# Autodesk Inventor assembly: Head
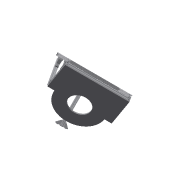
[picture p0: Inventor's stored thumbnail of the model, 180x180]
Saved by Autodesk Inventor 2014 SP1 (Build 180222100, 222)
## iProperties
Created: 2015-02-11
Part Number: Head
Document SubType Name: Assembly
Designer: Simen
Author: Simen
## Documents named in this file (9)
- C:\Users\Simen\Documents\git\Eit\skjellet\Head2.iam
- C:\Users\Simen\Documents\git\Eit\skjellet\HBL45TS6hbl45ts6.ipt
- C:\Users\Simen\Documents\git\Eit\skjellet\KHFS5_2020_386.ipt
- C:\Users\Simen\Documents\git\Eit\skjellet\KHFS5_2020_391.ipt
- C:\Users\Simen\Documents\git\Eit\skjellet\KHFS5_2020_220.ipt
- C:\Users\Simen\Documents\git\Eit\skjellet\frontPlate_half.ipt
- C:\Users\Simen\Documents\git\Eit\skjellet\jorneFester.iam
- C:\Users\Simen\Documents\git\Eit\skjellet\KHFS5_2020_426.ipt
- C:\Users\Simen\Documents\git\Eit\skjellet\KHFS5_2020_330.ipt
## Components (22 placed, 4 different names)
1. HBL45TS6hbl45ts6:2 — Mate:41, Flush:39, Mate:44, Mate:74, Mate:75, Flush:59
2. KHFS5-2020-4000:17 — Flush:64, Mate:83, Flush:65, Flush:66, Flush:67, Flush:68, Mate:84, Flush:83
3. KHFS5-2020-4000:18 — Mate:41, Flush:39, Mate:44, Mate:124, Flush:119, Flush:120, Mate:126, Flush:121
4. KHFS5-2020-4000:19 — Mate:81, Flush:63, Mate:82, Mate:116, Flush:115
5. KHFS5-2020-4000:34 — Mate:74, Mate:75, Flush:59, Flush:64, Flush:67, Flush:68, Mate:84, Flush:82, Mate:123, Mate:125
6. HBL45TS6hbl45ts6:3 — Mate:81, Flush:63
7. KHFS5-2020-4000:35 — Mate:82, Mate:83, Flush:65, Flush:66, Mate:93, Mate:117, Flush:116, Mate:119
8. frontPlate_half:1 — Mate:93, Flush:82, Flush:83
9. jorneFester:7 [sub-assembly] — Mate:129, Mate:131, Flush:124
10. jorneFester:5 [sub-assembly] — Mate:134, Mate:136, Flush:126, Flush:127, Flush:128, Mate:137, Flush:129
11. jorneFester:4 [sub-assembly] — Mate:128, Mate:132, Flush:123
12. jorneFester:2 [sub-assembly] — Mate:133, Mate:134, Flush:125, Flush:126, Mate:137, Mate:138
13. jorneFester:1 [sub-assembly] — Mate:133, Mate:135, Flush:127, Mate:139
14. jorneFester:3 [sub-assembly] — Mate:135, Mate:136, Flush:125, Flush:128
15. HBL45TS6hbl45ts6:4 — Mate:116, Flush:115
16. KHFS5-2020-4000:48 — Mate:118, Mate:119
17. jorneFester:8 [sub-assembly] — Mate:117, Flush:116, Mate:118
18. HBL45TS6hbl45ts6:5 — Mate:124, Flush:119
19. KHFS5-2020-4000:49 — Flush:118, Mate:125
20. jorneFester:9 [sub-assembly] — Mate:123, Flush:118
21. KHFS5-2020-4000:50 — Flush:120, Mate:126, Flush:121, Mate:128, Mate:129, Mate:130, Flush:122, Flush:123, Flush:124
22. KHFS5-2020-4000:51 — Mate:130, Flush:122, Mate:131, Mate:132, Mate:138, Mate:139, Flush:129
## Relationships (63: Mate 36, Flush 27)
- Mate:41: HBL45TS6hbl45ts6:2 ↔ KHFS5-2020-4000:18
- Flush:39: HBL45TS6hbl45ts6:2 ↔ KHFS5-2020-4000:18
- Mate:44: HBL45TS6hbl45ts6:2 ↔ KHFS5-2020-4000:18
- Mate:74: HBL45TS6hbl45ts6:2 ↔ KHFS5-2020-4000:34
- Mate:75: HBL45TS6hbl45ts6:2 ↔ KHFS5-2020-4000:34
- Flush:59: HBL45TS6hbl45ts6:2 ↔ KHFS5-2020-4000:34
- [Mate]: HBL45TS6hbl45ts6:3 ↔ KHFS5-2020-4000:35
- [Mate]: HBL45TS6hbl45ts6:3 ↔ KHFS5-2020-4000:35
- [Flush]: HBL45TS6hbl45ts6:3 ↔ KHFS5-2020-4000:35
- Mate:81: KHFS5-2020-4000:19 ↔ HBL45TS6hbl45ts6:3
- Flush:63: KHFS5-2020-4000:19 ↔ HBL45TS6hbl45ts6:3
- Mate:82: KHFS5-2020-4000:19 ↔ KHFS5-2020-4000:35
- Flush:64: KHFS5-2020-4000:17 ↔ KHFS5-2020-4000:34
- Mate:83: KHFS5-2020-4000:17 ↔ KHFS5-2020-4000:35
- Flush:65: KHFS5-2020-4000:17 ↔ KHFS5-2020-4000:35
- Flush:66: KHFS5-2020-4000:17 ↔ KHFS5-2020-4000:35
- Flush:67: KHFS5-2020-4000:17 ↔ KHFS5-2020-4000:34
- Flush:68: KHFS5-2020-4000:17 ↔ KHFS5-2020-4000:34
- Mate:84: KHFS5-2020-4000:17 ↔ KHFS5-2020-4000:34
- Mate:93: KHFS5-2020-4000:35 ↔ frontPlate_half:1
- Flush:82: KHFS5-2020-4000:34 ↔ frontPlate_half:1
- Flush:83: KHFS5-2020-4000:17 ↔ frontPlate_half:1
- [Mate]: HBL45TS6hbl45ts6:4 ↔ KHFS5-2020-4000:48
- [Mate]: HBL45TS6hbl45ts6:4 ↔ KHFS5-2020-4000:48
- [Flush]: HBL45TS6hbl45ts6:4 ↔ KHFS5-2020-4000:48
- Mate:116: KHFS5-2020-4000:19 ↔ HBL45TS6hbl45ts6:4
- Flush:115: KHFS5-2020-4000:19 ↔ HBL45TS6hbl45ts6:4
- Mate:117: KHFS5-2020-4000:35 ↔ jorneFester:8
- Flush:116: KHFS5-2020-4000:35 ↔ jorneFester:8
- Mate:118: KHFS5-2020-4000:48 ↔ jorneFester:8
- Mate:119: KHFS5-2020-4000:35 ↔ KHFS5-2020-4000:48
- [Mate]: HBL45TS6hbl45ts6:5 ↔ KHFS5-2020-4000:49
- [Mate]: HBL45TS6hbl45ts6:5 ↔ KHFS5-2020-4000:49
- [Flush]: HBL45TS6hbl45ts6:5 ↔ KHFS5-2020-4000:49
- [Mate]: KHFS5-2020-4000:49 ↔ jorneFester:9
- Mate:123: KHFS5-2020-4000:34 ↔ jorneFester:9
- Flush:118: KHFS5-2020-4000:49 ↔ jorneFester:9
- Mate:124: KHFS5-2020-4000:18 ↔ HBL45TS6hbl45ts6:5
- Flush:119: KHFS5-2020-4000:18 ↔ HBL45TS6hbl45ts6:5
- Mate:125: KHFS5-2020-4000:34 ↔ KHFS5-2020-4000:49
- Flush:120: KHFS5-2020-4000:18 ↔ KHFS5-2020-4000:50
- Mate:126: KHFS5-2020-4000:18 ↔ KHFS5-2020-4000:50
- Flush:121: KHFS5-2020-4000:18 ↔ KHFS5-2020-4000:50
- Mate:128: jorneFester:4 ↔ KHFS5-2020-4000:50
- Mate:129: jorneFester:7 ↔ KHFS5-2020-4000:50
- Mate:130: KHFS5-2020-4000:50 ↔ KHFS5-2020-4000:51
- Flush:122: KHFS5-2020-4000:50 ↔ KHFS5-2020-4000:51
- Mate:131: jorneFester:7 ↔ KHFS5-2020-4000:51
- Mate:132: jorneFester:4 ↔ KHFS5-2020-4000:51
- Flush:123: jorneFester:4 ↔ KHFS5-2020-4000:50
- Flush:124: jorneFester:7 ↔ KHFS5-2020-4000:50
- Mate:133: jorneFester:2 ↔ jorneFester:1
- Mate:134: jorneFester:5 ↔ jorneFester:2
- Mate:135: jorneFester:1 ↔ jorneFester:3
- Mate:136: jorneFester:5 ↔ jorneFester:3
- Flush:125: jorneFester:2 ↔ jorneFester:3
- Flush:126: jorneFester:5 ↔ jorneFester:2
- Flush:127: jorneFester:5 ↔ jorneFester:1
- Flush:128: jorneFester:5 ↔ jorneFester:3
- Mate:137: jorneFester:5 ↔ jorneFester:2
- Mate:138: jorneFester:2 ↔ KHFS5-2020-4000:51
- Mate:139: jorneFester:1 ↔ KHFS5-2020-4000:51
- Flush:129: jorneFester:5 ↔ KHFS5-2020-4000:51
## Named parameters: d171_d163 = 0 mm, d172_d164 = 0 mm, d173_d165 = 0 mm, d288_d171_d163 = 0 mm, d289_d172_d164 = 0 mm, d290_d173_d165 = 0 mm, d298_d296 = 0 mm, d299_d288_d171_d163 = 0 mm, d300_d289_d172_d164 = 0 mm, d301_d290_d173_d165 = 0 mm
